# Autodesk Inventor assembly: правый привод_MIR
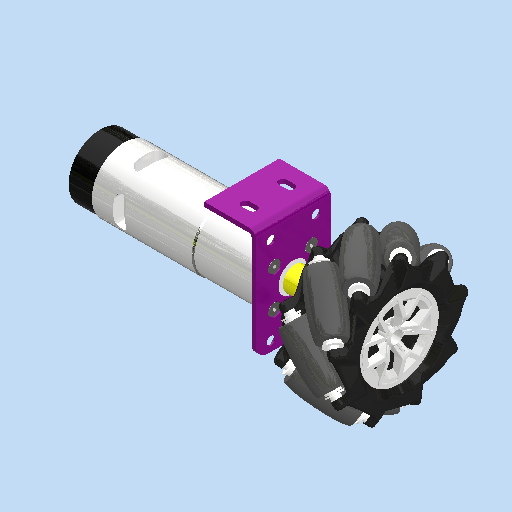
[picture p0: Inventor's stored thumbnail of the model, 512x512]
Saved by Autodesk Inventor 2025 (Build 290162000, 162)
## iProperties
Created: 2025-02-16
Part Number: правый привод_MIR
Document SubType Name: Assembly
Designer: volko
Author: volko
## Documents named in this file (8)
- C:\Users\volko\Desktop\диплом\Модели\детали\левый привод.iam
- C:\Users\volko\Desktop\диплом\Модели\детали\CHP-42GP-775 ABHL_MIR.ipt
- C:\Users\volko\Desktop\диплом\Модели\детали\кронштейн_MIR.ipt
- C:\Users\volko\Desktop\диплом\Модели\детали\переходная втулка_MIR.ipt
- C:\Users\volko\Desktop\диплом\Модели\Mecanum wheel - left\Mecanum wheel - left.iam
- C:\Users\volko\Desktop\диплом\Модели\детали\стандартные изделия\ru-RU\DIN 7991(2)\DIN 7991 - M4x8.ipt
- C:\Users\volko\Desktop\диплом\Модели\детали\стандартные изделия\ru-RU\ISO 7380-1\ISO 7380-1 - M4 x 25.ipt
- C:\Users\volko\Desktop\диплом\Модели\детали\стандартные изделия\ru-RU\DIN 913\DIN 913 - M3 x 4.ipt
## Components (10 placed, 7 different names)
1. CHP-42GP-775 ABHL_MIR:1 — Совмещение:1, Совмещение:2, Заподлицо:1, Совмещение:3, Совмещение:4, Совмещение:5, Совмещение:7, Совмещение:11, Совмещение:21
2. кронштейн_MIR:1 — Совмещение:5, Совмещение:7, Совмещение:11, Совмещение:13, Совмещение:14, Совмещение:15, Совмещение:16
3. переходная втулка_MIR:1 — Совмещение:3, Совмещение:4, Совмещение:8, Совмещение:9, Совмещение:10, Заподлицо:18, Совмещение:20
4. Mecanum wheel - left:1 [sub-assembly] — Совмещение:8, Совмещение:9, Совмещение:10, Совмещение:18, Совмещение:19
5. ISO 7380-1 M4 x 25:1 — Совмещение:18, Совмещение:19
6. DIN 913 M3 x 4:1 — Совмещение:20, Совмещение:21
7. DIN 7991 M4x8:1 — Совмещение:13
8. DIN 7991 M4x8:2 — Совмещение:14
9. DIN 7991 M4x8:3 — Совмещение:15
10. DIN 7991 M4x8:4 — Совмещение:16
## Relationships (20: Mate 18, Flush 2)
- Совмещение:1 [Mate]: CHP-42GP-775 ABHL_MIR:1
- Совмещение:2 [Mate]: CHP-42GP-775 ABHL_MIR:1
- Заподлицо:1 [Flush]: CHP-42GP-775 ABHL_MIR:1
- Совмещение:3 [Mate]: CHP-42GP-775 ABHL_MIR:1 ↔ переходная втулка_MIR:1
- Совмещение:4 [Mate]: CHP-42GP-775 ABHL_MIR:1 ↔ переходная втулка_MIR:1
- Совмещение:5 [Mate]: CHP-42GP-775 ABHL_MIR:1 ↔ кронштейн_MIR:1
- Совмещение:7 [Mate]: CHP-42GP-775 ABHL_MIR:1 ↔ кронштейн_MIR:1
- Совмещение:8 [Mate]: переходная втулка_MIR:1 ↔ Mecanum wheel - left:1
- Совмещение:9 [Mate]: переходная втулка_MIR:1 ↔ Mecanum wheel - left:1
- Совмещение:10 [Mate]: переходная втулка_MIR:1 ↔ Mecanum wheel - left:1
- Совмещение:11 [Mate]: CHP-42GP-775 ABHL_MIR:1 ↔ кронштейн_MIR:1
- Совмещение:13 [Mate]: кронштейн_MIR:1 ↔ DIN 7991 M4x8:1
- Совмещение:14 [Mate]: кронштейн_MIR:1 ↔ DIN 7991 M4x8:2
- Совмещение:15 [Mate]: кронштейн_MIR:1 ↔ DIN 7991 M4x8:3
- Совмещение:16 [Mate]: кронштейн_MIR:1 ↔ DIN 7991 M4x8:4
- Заподлицо:18 [Flush]: переходная втулка_MIR:1
- Совмещение:18 [Mate]: Mecanum wheel - left:1 ↔ ISO 7380-1 M4 x 25:1
- Совмещение:19 [Mate]: Mecanum wheel - left:1 ↔ ISO 7380-1 M4 x 25:1
- Совмещение:20 [Mate]: переходная втулка_MIR:1 ↔ DIN 913 M3 x 4:1
- Совмещение:21 [Mate]: CHP-42GP-775 ABHL_MIR:1 ↔ DIN 913 M3 x 4:1
